# Autodesk Inventor assembly: C-MLG9-235
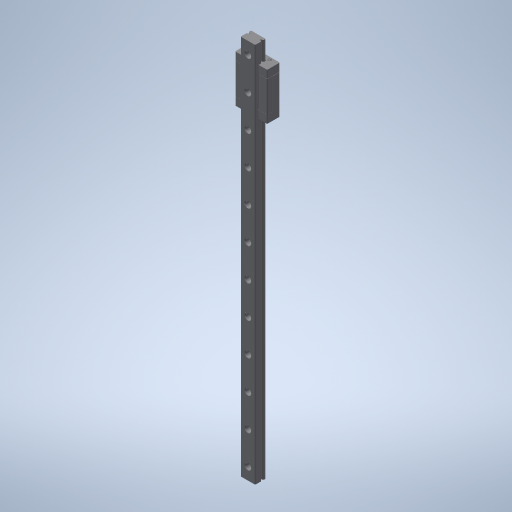
[picture p0: Inventor's stored thumbnail of the model, 512x512]
Saved by Autodesk Inventor 2024.1 (Build 281209000, 209)
## iProperties
Category: PARTsolutions
Company: MISUMI
Created: 2023-08-25
Part Number: C-MLG9-235
Catalog Web Link: www.cadenas.de
Description: C-MLG, C-MLGL, E-GMLG-Economy Miniature Liner Guides - Standard Type
Vendor: MISUMI
Document SubType Name: Assembly
Designer: psAdmin
Manufacturer: MISUMI
Mass: 14.5892 g
Surface Area: 112.679 cm^2
Volume: 14.5892 cm^3
PSOL_IDENT_0: {$CADENAS_DATA/23d-libs/misumi/metric/06_linear_guides/c_mlg_asmtab.prj},197 {VTYP=3D},{STYP=ASSTAB}
PSOL_IDENT_1: ,{NB=C-MLG9-235},{LINA=C-MLG9-235},{NN=C-MLG, C-MLGL, E-GMLG},{DATE=14.07.2023 05:46:03},{GEOMDATE=0
PSOL_IDENT_2: 1.12.2022 04:31:45},{VERSION=},{LINEID=20},{WBVAR=ST,LT,L},{WBNUMERIC=L}  {NB=C-MLG9-235},{LINA=C-ML
PSOL_IDENT_3: G9-235},{KT=DUMMY},{PN=C-MLG9-235},{ST=1},{LT=S},{TYPE=C-MLG},{WR=9},{L=235},{LALG=[35,55,75,95,115,
PSOL_IDENT_4: 135,155,175,195,215,235,255,275]},{LALG1=[35,55,75,95,115,135,155,175,195,215,235,255,275]},{LALG2=[
PSOL_IDENT_5: 36:54/1],[56:74/1],[76:94/1],[96:114/1],[116:134/1],[136:154/1],[156:174/1],[176:194/1],[196:214/1],
PSOL_IDENT_6: [216:234/1],[236:254/1],[256:274/1],[276:355/1]},{LPN=-235},{H=10},{H1=2.0},{N=5.5},{W=20},{B=15},{B
PSOL_IDENT_7: 1=2.5},{C=10},{L1=18.9},{L2=29.60},{GNN=Dia.1.4},{M=3},{LL=3.0},{ML=M3x3},{H2=1.8},{HRR=6.5},{D=6.0}
PSOL_IDENT_8: ,{HH=3.5},{DD=3.5},{P=20},{M1=12},{E=7.5},{NA=11},{PPATH=c_mlg/c_mlg_asmtpl.prj},{LTALG='S', 'L Sele
PSOL_IDENT_9: ctable Type', 'C', 'L Configurable Type'},{LALG3=[35:355/1]}
NB: C-MLG9-235
NN: C-MLG, C-MLGL, E-GMLG
NT: Economy Miniature Liner Guides - Standard Type
NBSYN: $PN.
LINA: C-MLG9-235
CATALOG: Misumi
PN: C-MLG9-235
ST: No Surface Treatment
LT: L Selectable Type
WR: 9
L: 235
H: 10
H1: 2
N: 5.5
W: 20
B: 15
B1: 2.5
C: 10
L1: 18.9
L2: 29.6
GNN: Dia.1.4
ML: M3x3
H2: 1.8
HRR: 6.5
D: 6
HH: 3.5
DD: 3.5
P: 20
E: 7.5
SUPPLIER: MISUMI
ARTICLENO: C-MLG9-235
BOMINFO: C-MLG9-235
CREATOR: CADENAS GmbH
Title: C-MLG9-235
Author: Cadenas PARTsolutions
Comments: Economy Miniature Liner Guides - Standard Type
## Documents named in this file (3)
- C:\Users\haruy\OneDrive - Kyushu University\KURT_工房共有\2023~2024\ハード\CAD\2024NHK\000_parts\スライダー\C-MLG9-235\AIS2022\C-MLG9-235.iam
- C:\Users\haruy\OneDrive - Kyushu University\KURT_工房共有\2023~2024\ハード\CAD\2024NHK\000_parts\スライダー\C-MLG9-235\AIS2022\C-MLG9-235_r.ipt
- C:\Users\haruy\OneDrive - Kyushu University\KURT_工房共有\2023~2024\ハード\CAD\2024NHK\000_parts\スライダー\C-MLG9-235\AIS2022\C-MLGB9.ipt
## Components (2 placed, 2 different names)
1. C-MLG9-235_r:1 — to_body_Z@1 <-> to_rail_Z@2, スライダ:1
2. C-MLGB9:1 — to_body_Z@1 <-> to_rail_Z@2, スライダ:1
## Relationships (2: Mate 1, TranslationJoint 1)
- to_body_Z@1 <-> to_rail_Z@2 [Mate]: C-MLG9-235_r:1 ↔ C-MLGB9:1
- スライダ:1 [TranslationJoint] (0.1 mm): C-MLG9-235_r:1 ↔ C-MLGB9:1
